# Autodesk Inventor assembly: 67498-shock absorber
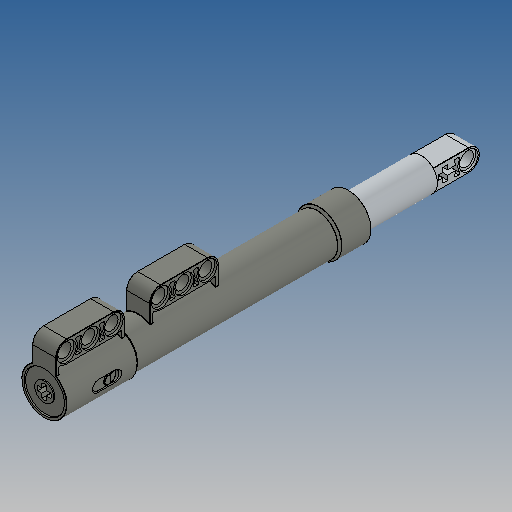
[picture p0: Inventor's stored thumbnail of the model, 512x512]
Saved by Autodesk Inventor 2025 (Build 290162010, 162A)
## iProperties
Created: 2024-12-01
Part Number: 67498-shock absorber
Material: Generisch
Document SubType Name: Assembly
Designer: hp.muther
Author: hp.muther
## Documents named in this file (3)
- D:\Inventor\Projekte\Muther\LEGO Technic\LEGO Pieces\67498-shock absorber.iam
- D:\Inventor\Projekte\Muther\LEGO Technic\LEGO Pieces\_Einzelteile zu Baugruppen\67498_01.ipt
- D:\Inventor\Projekte\Muther\LEGO Technic\LEGO Pieces\_Einzelteile zu Baugruppen\67498_02.ipt
## Components (2 placed, 2 different names)
1. 67498_01:1 — Passend:1, Passend:2, Passend:3
2. 67498_02:1 — Passend:1, Passend:2, Passend:3
## Relationships (3: Mate 3)
- Passend:1 [Mate]: 67498_01:1 ↔ 67498_02:1
- Passend:2 [Mate]: 67498_01:1 ↔ 67498_02:1
- Passend:3 [Mate]: 67498_01:1 ↔ 67498_02:1
